# Autodesk Inventor assembly: Level 2 Ring Assembly
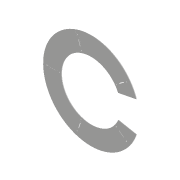
[picture p0: Inventor's stored thumbnail of the model, 180x180]
Saved by Autodesk Inventor 2020 (Build 240168000, 168)
## iProperties
Created: 2020-08-03
Part Number: Level 2 Ring Assembly
Document SubType Name: Assembly
Designer: Dan Wikman
Author: Dan Wikman
## Documents named in this file (5)
- C:\Users\Dan Wikman\OneDrive\University Life\2020, Semester 1\METR4900 Honours Thesis\PROTOTYPE V2\Level 2 Ring Assembly.iam
- C:\Users\Dan Wikman\OneDrive\University Life\2020, Semester 1\METR4900 Honours Thesis\PROTOTYPE V2\Level 2a - V2.ipt
- C:\Users\Dan Wikman\OneDrive\University Life\2020, Semester 1\METR4900 Honours Thesis\PROTOTYPE V2\Level 2b - V2.ipt
- C:\Users\Dan Wikman\OneDrive\University Life\2020, Semester 1\METR4900 Honours Thesis\PROTOTYPE V2\Level 2c - V2.ipt
- C:\Users\Dan Wikman\OneDrive\University Life\2020, Semester 1\METR4900 Honours Thesis\PROTOTYPE V2\Level 2d - V2.ipt
## Components (4 placed, 4 different names)
1. Level 2a - V2:1 — Flush:1, Mate:1, Mate:4
2. Level 2b - V2:1 — Flush:1, Flush:2, Mate:1, Mate:2, Mate:4, Mate:5
3. Level 2c - V2:1 — Flush:2, Flush:3, Mate:2, Mate:3, Mate:5, Mate:6
4. Level 2d - V2:1 — Flush:3, Mate:3, Mate:6
## Relationships (9: Mate 6, Flush 3)
- Flush:1: Level 2a - V2:1 ↔ Level 2b - V2:1
- Flush:2: Level 2b - V2:1 ↔ Level 2c - V2:1
- Flush:3: Level 2c - V2:1 ↔ Level 2d - V2:1
- Mate:1: Level 2a - V2:1 ↔ Level 2b - V2:1
- Mate:2: Level 2b - V2:1 ↔ Level 2c - V2:1
- Mate:3: Level 2c - V2:1 ↔ Level 2d - V2:1
- Mate:4: Level 2a - V2:1 ↔ Level 2b - V2:1
- Mate:5: Level 2b - V2:1 ↔ Level 2c - V2:1
- Mate:6: Level 2c - V2:1 ↔ Level 2d - V2:1
